# Autodesk Inventor assembly: Motor Mount Assy
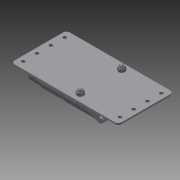
[picture p0: Inventor's stored thumbnail of the model, 180x180]
Saved by Autodesk Inventor 2014 (Build 180170000, 170)
## iProperties
Created: 2015-01-20
Part Number: Motor Mount Assy
Document SubType Name: Assembly
Designer: chappelled
Author: chappelled
## Documents named in this file (7)
- C:\Users\chappelled\Documents\Inventor\Claw\Motor Mount Assy.iam
- C:\Users\chappelled\Documents\Inventor\Claw\Motor Mount.ipt
- C:\Users\chappelled\Documents\Inventor\Claw\Imported Components\PG71BracketAM-2197\PG71BracketAM-2197.ipt
- C:\Users\chappelled\Documents\Inventor\Claw\Imported Components\PG-71-am-0914\PG-71-am-0914.ipt
- C:\Users\chappelled\Documents\Inventor\Content Center Files\R2014\en-US\JIS B 1176\JIS B 1176 - M4 x 6.ipt
- C:\Users\chappelled\Documents\Inventor\Claw\Motor Mount Assy\Design Accelerator\Bolted Connection1.iam
- C:\Users\chappelled\Documents\Inventor\Claw\Motor Mount Assy\Design Accelerator\Bolted Connection2.iam
## Components (9 placed, 5 different names)
1. Motor Mount:1 — Mate:2, Mate:3, Mate:14, Mate:16
2. PG71BracketAM-2197:1 — Mate:2, Mate:3, Mate:4, Mate:5, Mate:6, Mate:7, Mate:8, Mate:9, Mate:10, Mate:11, Mate:12, Mate:13, Mate:14, Mate:15, Mate:17, Mate:18
3. PG-71-am-0914:1 — Mate:4, Mate:5
4. JIS B 1176 - Metric M4 x 6:1 — Mate:6, Mate:7
5. JIS B 1176 - Metric M4 x 6:2 — Mate:8, Mate:9
6. JIS B 1176 - Metric M4 x 6:3 — Mate:10, Mate:11
7. JIS B 1176 - Metric M4 x 6:4 — Mate:12, Mate:13
8. Bolted Connection:1 [sub-assembly] — Mate:15, Mate:16
9. Bolted Connection:2 [sub-assembly] — Mate:17, Mate:18
## Relationships (17: Mate 17)
- Mate:2: Motor Mount:1 ↔ PG71BracketAM-2197:1
- Mate:3: Motor Mount:1 ↔ PG71BracketAM-2197:1
- Mate:4: PG71BracketAM-2197:1 ↔ PG-71-am-0914:1
- Mate:5: PG71BracketAM-2197:1 ↔ PG-71-am-0914:1
- Mate:6: PG71BracketAM-2197:1 ↔ JIS B 1176 - Metric M4 x 6:1
- Mate:7: PG71BracketAM-2197:1 ↔ JIS B 1176 - Metric M4 x 6:1
- Mate:8: PG71BracketAM-2197:1 ↔ JIS B 1176 - Metric M4 x 6:2
- Mate:9: PG71BracketAM-2197:1 ↔ JIS B 1176 - Metric M4 x 6:2
- Mate:10: PG71BracketAM-2197:1 ↔ JIS B 1176 - Metric M4 x 6:3
- Mate:11: PG71BracketAM-2197:1 ↔ JIS B 1176 - Metric M4 x 6:3
- Mate:12: PG71BracketAM-2197:1 ↔ JIS B 1176 - Metric M4 x 6:4
- Mate:13: PG71BracketAM-2197:1 ↔ JIS B 1176 - Metric M4 x 6:4
- Mate:14: Motor Mount:1 ↔ PG71BracketAM-2197:1
- Mate:15: PG71BracketAM-2197:1 ↔ Bolted Connection:1
- Mate:16: Motor Mount:1 ↔ Bolted Connection:1
- Mate:17: PG71BracketAM-2197:1 ↔ Bolted Connection:2
- Mate:18: PG71BracketAM-2197:1 ↔ Bolted Connection:2
